# Autodesk Inventor assembly: Asem
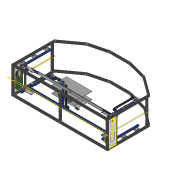
[picture p0: Inventor's stored thumbnail of the model, 180x180]
Saved by Autodesk Inventor 2020 (Build 240168000, 168)
## iProperties
Created: 2021-02-24
Part Number: Asem
Document SubType Name: Assembly
Designer: magnarecta
Author: magnarecta
## Documents named in this file (10)
- D:\Document\Github\Eto_Project\Hardware\Asem\Asem.iam
- D:\Document\Github\Eto_Project\Hardware\Asem\CCM_Unit.iam
- D:\Document\Github\Eto_Project\Hardware\Asem\Display_Unit.iam
- D:\Document\Github\Eto_Project\Hardware\Parts\Grabcad\nema-23-stepper-motors-driver-1.snapshot.7\DM542T Digital Stepper Drive.ipt
- D:\Document\Github\Eto_Project\Hardware\Parts\Grabcad\mean-well-lrs-350-24-1.snapshot.3\meanwell_lrs-350-24_UPDATED.ipt
- D:\Document\Github\Eto_Project\Hardware\Parts\Grabcad\ac-power-switch-assembly-1.snapshot.2\AC Power Switch Assy.iam
- D:\Document\Github\Eto_Project\Hardware\Parts\MISUMI_FRAMES\model_ver4\1208.iam
- D:\Document\Github\Eto_Project\Hardware\Parts\Laser_Cut\Cut_A.ipt
- D:\Document\Github\Eto_Project\Hardware\Parts\Laser_Cut\Cut_B.ipt
- D:\Document\Github\Eto_Project\Hardware\Parts\Grabcad\mks-base-1-4-1.snapshot.2\MKS 1.4 Board.ipt
## Components (16 placed, 9 different names)
1. CCM_Unit:1 [sub-assembly] — 挿入:1, 挿入:2, フラッシュ:5, メイト:4, フラッシュ:6
2. Display_Unit:1 [sub-assembly] — 挿入:1, 挿入:2
3. meanwell_lrs-350-24_UPDATED:1 — 挿入:4, メイト:17
4. AC Power Switch Assy:1 [sub-assembly] — フラッシュ:3, 挿入:5
5. AC Power Switch Assy:2 [sub-assembly] — フラッシュ:3, 挿入:6, メイト:18
6. 1208:1 [sub-assembly] — メイト:1, メイト:2, メイト:3, フラッシュ:5, メイト:4, フラッシュ:6, メイト:9, メイト:10, 角度:1, メイト:13, メイト:14, メイト:15, メイト:16
7. Cut_B:1 — メイト:9, メイト:10, 挿入:3, メイト:11, メイト:12, メイト:13
8. MKS 1.4 Board:1 — メイト:11, 角度:1, メイト:12
9. Cut_A:1 — メイト:14, メイト:15, メイト:16, 挿入:4, メイト:17, 挿入:5, 挿入:6, メイト:18
10. DM542T Digital Stepper Drive:1
11. DM542T Digital Stepper Drive:2
12. DM542T Digital Stepper Drive:3
13. DM542T Digital Stepper Drive:4
14. DM542T Digital Stepper Drive:5
15. DM542T Digital Stepper Drive:6
16. DM542T Digital Stepper Drive:7 — 挿入:3
## Component patterns: (7 elements, first: DM542T Digital Stepper Drive:1)
## Relationships (24: Mate 14, Insert 6, Flush 3, Angle 1)
- 挿入:1 [Insert]: CCM_Unit:1 ↔ Display_Unit:1
- フラッシュ:3 [Flush]: AC Power Switch Assy:1 ↔ AC Power Switch Assy:2
- 挿入:2 [Insert]: CCM_Unit:1 ↔ Display_Unit:1
- メイト:1 [Mate]: 1208:1
- メイト:2 [Mate] (-1400 mm): 1208:1
- メイト:3 [Mate] (355 mm): 1208:1
- フラッシュ:5 [Flush]: CCM_Unit:1 ↔ 1208:1
- メイト:4 [Mate]: CCM_Unit:1 ↔ 1208:1
- フラッシュ:6 [Flush]: CCM_Unit:1 ↔ 1208:1
- メイト:9 [Mate] (1 mm): 1208:1 ↔ Cut_B:1
- メイト:10 [Mate] (1 mm): 1208:1 ↔ Cut_B:1
- 挿入:3 [Insert]: Cut_B:1 ↔ DM542T Digital Stepper Drive:7
- メイト:11 [Mate] (5 mm): Cut_B:1 ↔ MKS 1.4 Board:1
- 角度:1 [Angle] (0 deg): 1208:1 ↔ MKS 1.4 Board:1
- メイト:12 [Mate]: Cut_B:1 ↔ MKS 1.4 Board:1
- メイト:13 [Mate] (-5 mm): 1208:1 ↔ Cut_B:1
- メイト:14 [Mate] (-5 mm): 1208:1 ↔ Cut_A:1
- メイト:15 [Mate] (1 mm): 1208:1 ↔ Cut_A:1
- メイト:16 [Mate] (1 mm): 1208:1 ↔ Cut_A:1
- 挿入:4 [Insert]: meanwell_lrs-350-24_UPDATED:1 ↔ Cut_A:1
- メイト:17 [Mate]: meanwell_lrs-350-24_UPDATED:1 ↔ Cut_A:1
- 挿入:5 [Insert]: AC Power Switch Assy:1 ↔ Cut_A:1
- 挿入:6 [Insert]: AC Power Switch Assy:2 ↔ Cut_A:1
- メイト:18 [Mate]: AC Power Switch Assy:2 ↔ Cut_A:1
